# Autodesk Inventor assembly: Base
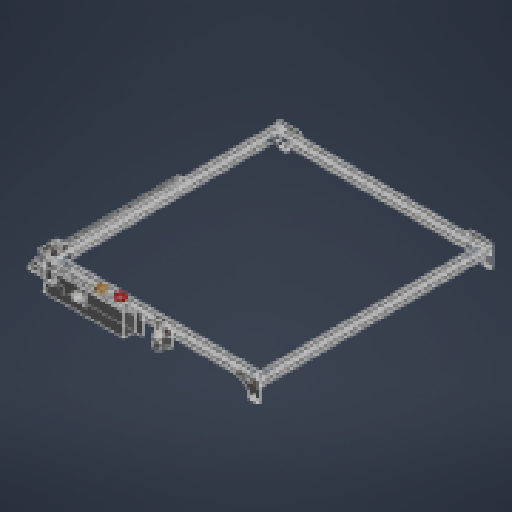
[picture p0: Inventor's stored thumbnail of the model, 512x512]
Saved by Autodesk Inventor 2025 (Build 290162000, 162)
## iProperties
Created: 2024-11-17
Part Number: Base
Document SubType Name: Assembly
Designer: Admin
Author: Admin
Revision Number: ANY
## Documents named in this file (23)
- V:\INVENTOR\laser\ortur\ortur_laser_master_s2_information\3D model\ortur_s2\Base.iam
- V:\INVENTOR\laser\ortur\ortur_laser_master_s2_information\3D model\ortur_s2\plain washer 6902 type abc_din_DIN 6902-A5.5.ipt
- V:\INVENTOR\laser\ortur\ortur_laser_master_s2_information\3D model\ortur_s2\Vis cruci_DIN EN ISO 7045 - M5 x 10 - Z - 10N.ipt
- V:\INVENTOR\laser\ortur\ortur_laser_master_s2_information\3D model\ortur_s2\Vis cruci_DIN EN ISO 7045 - M5 x 30 - Z - 30N.ipt
- V:\INVENTOR\laser\ortur\ortur_laser_master_s2_information\3D model\ortur_s2\Vis cruci_DIN EN ISO 7045 - M2 x 10 - Z - 10N.ipt
- V:\INVENTOR\laser\ortur\ortur_laser_master_s2_information\3D model\ortur_s2\Profilé 540mm.ipt
- V:\INVENTOR\laser\ortur\ortur_laser_master_s2_information\3D model\ortur_s2\Profilé 460mm.ipt
- V:\INVENTOR\laser\ortur\ortur_laser_master_s2_information\3D model\ortur_s2\Pied.ipt
- V:\INVENTOR\laser\ortur\ortur_laser_master_s2_information\3D model\ortur_s2\Support capteur Y.ipt
- V:\INVENTOR\laser\ortur\ortur_laser_master_s2_information\3D model\ortur_s2\Microswitch Omron SS-5GL-F.ipt
- V:\INVENTOR\laser\ortur\ortur_laser_master_s2_information\3D model\ortur_s2\Panneau de controle.ipt
- V:\INVENTOR\laser\ortur\ortur_laser_master_s2_information\3D model\ortur_s2\connecteur 2x9.ipt
- V:\INVENTOR\laser\ortur\ortur_laser_master_s2_information\3D model\ortur_s2\connecteur 2x5.ipt
- V:\INVENTOR\laser\ortur\ortur_laser_master_s2_information\3D model\ortur_s2\PJ-102BH.ipt
- V:\INVENTOR\laser\ortur\ortur_laser_master_s2_information\3D model\ortur_s2\USB 2.0 Type B Connector Right Angle (Würth 61400416121).ipt
- V:\INVENTOR\laser\ortur\ortur_laser_master_s2_information\3D model\ortur_s2\RJ11_Female_Connector.ipt
- V:\INVENTOR\laser\ortur\ortur_laser_master_s2_information\3D model\ortur_s2\connecteur 2x3.ipt
- V:\INVENTOR\laser\ortur\ortur_laser_master_s2_information\3D model\ortur_s2\Support cale focus.ipt
- V:\INVENTOR\laser\ortur\ortur_laser_master_s2_information\3D model\ortur_s2\Cale focus.ipt
- V:\INVENTOR\laser\ortur\ortur_laser_master_s2_information\3D model\ortur_s2\Mousse pieds.ipt
- V:\INVENTOR\laser\ortur\ortur_laser_master_s2_information\3D model\ortur_s2\2020_int_L_joint___ _________.ipt
- V:\INVENTOR\laser\ortur\ortur_laser_master_s2_information\3D model\ortur_s2\Support chaine.ipt
- V:\INVENTOR\laser\ortur\ortur_laser_master_s2_information\3D model\ortur_s2\Chaine porte cable 1_350.ipt
## Components (46 placed, 46 different names)
1. plain washer 6902 type abc_din_DIN 6902-A5.5_199
2. Vis cruci_DIN EN ISO 7045 - M5 x 10 - Z - 10N_200
3. Vis cruci_DIN EN ISO 7045 - M5 x 30 - Z - 30N_201
4. plain washer 6902 type abc_din_DIN 6902-A5.5_202
5. plain washer 6902 type abc_din_DIN 6902-A5.5_203
6. Vis cruci_DIN EN ISO 7045 - M5 x 30 - Z - 30N_204
7. Vis cruci_DIN EN ISO 7045 - M5 x 10 - Z - 10N_205
8. Vis cruci_DIN EN ISO 7045 - M5 x 30 - Z - 30N_206
9. Vis cruci_DIN EN ISO 7045 - M5 x 10 - Z - 10N_207
10. Vis cruci_DIN EN ISO 7045 - M2 x 10 - Z - 10N_208
11. Vis cruci_DIN EN ISO 7045 - M2 x 10 - Z - 10N_209
12. Vis cruci_DIN EN ISO 7045 - M5 x 10 - Z - 10N_210
13. Vis cruci_DIN EN ISO 7045 - M5 x 10 - Z - 10N_211
14. Vis cruci_DIN EN ISO 7045 - M5 x 10 - Z - 10N_212
15. Vis cruci_DIN EN ISO 7045 - M5 x 10 - Z - 10N_213
16. Vis cruci_DIN EN ISO 7045 - M5 x 10 - Z - 10N_214
17. Vis cruci_DIN EN ISO 7045 - M5 x 10 - Z - 10N_215
18. Vis cruci_DIN EN ISO 7045 - M5 x 30 - Z - 30N_216
19. Profilé 540mm_217 — Symmetry:1
20. Profilé 460mm_218 — Symmetry:2
21. Profilé 540mm_219 — Symmetry:1
22. Profilé 460mm_220 — Symmetry:2
23. Pied_221
24. Pied_222
25. Pied_223
26. Support capteur Y_224
27. Microswitch Omron SS-5GL-F_225
28. Panneau de controle_226
29. connecteur 2x9_227
30. connecteur 2x5_228
31. PJ-102BH_229
32. USB 2.0 Type B Connector Right Angle (Würth 61400416121)_230
33. RJ11_Female_Connector_231
34. connecteur 2x3_232
35. Support cale focus_233
36. Cale focus_234
37. Mousse pieds_235
38. Mousse pieds_236
39. Mousse pieds_237
40. Mousse pieds_238
41. 2020_int_L_joint___ __________239
42. 2020_int_L_joint___ __________240
43. 2020_int_L_joint___ __________241
44. 2020_int_L_joint___ __________242
45. Support chaine_243
46. Chaine porte cable 1_350_244
## Relationships (2: Symmetry 2)
- Symmetry:1: Profilé 540mm_217 ↔ Profilé 540mm_219
- Symmetry:2: Profilé 460mm_218 ↔ Profilé 460mm_220
